# Autodesk Inventor assembly: Assembled Capsule
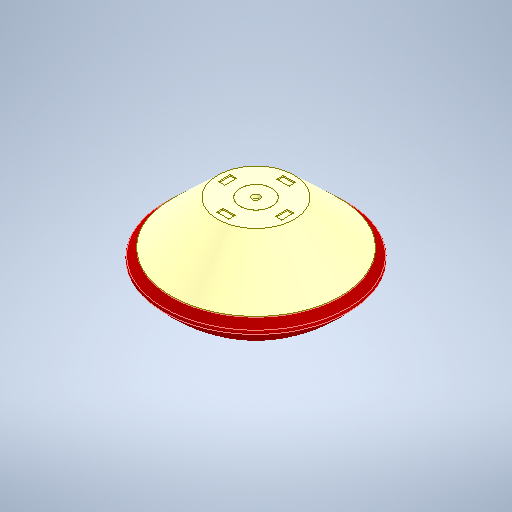
[picture p0: Inventor's stored thumbnail of the model, 512x512]
Saved by Autodesk Inventor 2026.2 (Build 302298000, 298)
## iProperties
Created: 2026-01-18
Part Number: Assembled Capsule
Document SubType Name: Assembly
Designer: daryu
Author: daryu
## Documents named in this file (13)
- C:\Users\daryu\Documents\RE entry capsule\Assembled Capsule.iam
- C:\Users\daryu\Documents\RE entry capsule\Front Shield TPS.ipt
- C:\Users\daryu\Documents\RE entry capsule\Front Shield Structure.ipt
- C:\Users\daryu\Documents\RE entry capsule\Energy Absorption Crush.ipt
- C:\Users\daryu\Documents\RE entry capsule\Internal Structure.ipt
- C:\Users\daryu\Documents\RE entry capsule\Back Cover.ipt
- C:\Users\daryu\Documents\RE entry capsule\Back Cover TPS.ipt
- C:\Users\daryu\Documents\RE entry capsule\Back Cover TPS seal.ipt
- C:\Users\daryu\Downloads\Lattices12x12x2\Lid(1 to 10)\Lid(1 to 10).ipt
- C:\Users\daryu\Downloads\Lattices12x12x2\Pod(1 to 10)\Pod(1 to 10).ipt
- C:\Users\daryu\Documents\Capsule idea.ipt
- C:\Users\daryu\Documents\RE entry capsule\Back Cover seal.ipt
- C:\Users\daryu\Documents\RE entry capsule\Mesh Assembly.iam
## Components (17 placed, 12 different names)
1. Front Shield TPS:1 — Mate:1, Mate:2, Angle:1
2. Front Shield Structure:1 — Mate:1, Mate:2, Mate:3, Mate:4
3. Energy Absorption Crush:1 — Mate:3, Mate:4, Mate:5, Mate:6, Insert:2
4. Internal Structure:1 — Mate:5, Mate:6, Mate:7, Mate:8
5. Back Cover:1 — Mate:7, Mate:8, Mate:9, Mate:10, Insert:10
6. Back Cover TPS:1 — Mate:9, Mate:10, Insert:1
7. Back Cover TPS seal:1 — Insert:1
8. Lid(1 to 10):1 — Insert:9
9. Pod(1 to 10):1 — Insert:2, Insert:3, Insert:4, Insert:5, Insert:6, Insert:7, Insert:8, Insert:9, Mate:11, Mate:12
10. Capsule idea:1 — Insert:3
11. Capsule idea:2 — Insert:4
12. Capsule idea:3 — Insert:6
13. Capsule idea:4 — Insert:7
14. Capsule idea:5 — Insert:5
15. Capsule idea:6 — Insert:8
16. Back Cover seal:1 — Insert:10
17. Mesh Assembly:1 [sub-assembly] — Mate:11, Mate:12, Angle:1
## Relationships (23: Mate 12, Insert 10, Angle 1)
- Mate:1: Front Shield TPS:1 ↔ Front Shield Structure:1
- Mate:2 (0.706 mm): Front Shield TPS:1 ↔ Front Shield Structure:1
- Mate:3: Front Shield Structure:1 ↔ Energy Absorption Crush:1
- Mate:4 (-10.118 mm): Front Shield Structure:1 ↔ Energy Absorption Crush:1
- Mate:5: Energy Absorption Crush:1 ↔ Internal Structure:1
- Mate:6 (-3.031 mm): Energy Absorption Crush:1 ↔ Internal Structure:1
- Mate:7: Internal Structure:1 ↔ Back Cover:1
- Mate:8: Internal Structure:1 ↔ Back Cover:1
- Mate:9: Back Cover:1 ↔ Back Cover TPS:1
- Mate:10: Back Cover:1 ↔ Back Cover TPS:1
- Insert:1: Back Cover TPS:1 ↔ Back Cover TPS seal:1
- Insert:2: Energy Absorption Crush:1 ↔ Pod(1 to 10):1
- Insert:3: Pod(1 to 10):1 ↔ Capsule idea:1
- Insert:4: Pod(1 to 10):1 ↔ Capsule idea:2
- Insert:5: Pod(1 to 10):1 ↔ Capsule idea:5
- Insert:6: Pod(1 to 10):1 ↔ Capsule idea:3
- Insert:7: Pod(1 to 10):1 ↔ Capsule idea:4
- Insert:8: Pod(1 to 10):1 ↔ Capsule idea:6
- Insert:9: Lid(1 to 10):1 ↔ Pod(1 to 10):1
- Insert:10: Back Cover:1 ↔ Back Cover seal:1
- Mate:11: Pod(1 to 10):1 ↔ Mesh Assembly:1
- Mate:12: Pod(1 to 10):1 ↔ Mesh Assembly:1
- Angle:1 (83 deg): Front Shield TPS:1 ↔ Mesh Assembly:1
